# Autodesk Inventor assembly: fourbarintakebearing_MIR_MIR1_MIR1_MIR
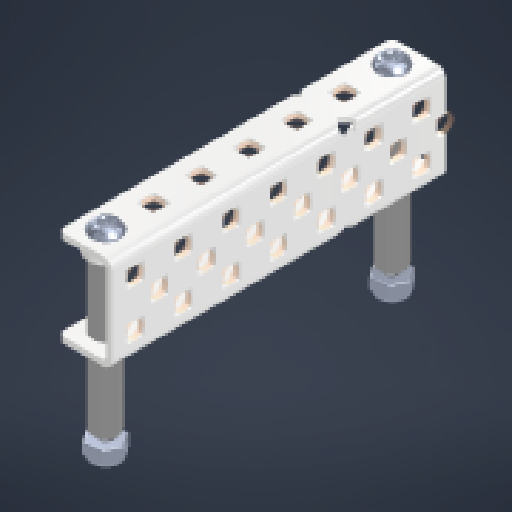
[picture p0: Inventor's stored thumbnail of the model, 512x512]
Saved by Autodesk Inventor 2023 (Build 270158000, 158)
## iProperties
Created: 2023-08-08
Part Number: fourbarintakebearing_MIR_MIR1_MIR1_MIR
Document SubType Name: Assembly
Designer: srbel
Author: srbel
## Documents named in this file (9)
- C:\CAD\OverUnderCAD\Drive\fourbarintakebearing_MIR_MIR1_MIR1_MIR.iam
- C:\CAD\OverUnderCAD\VEX-CAD-Inventor-1.4.0\Structure\C Channel\Aluminum 1x2x1\Alu C 1x2x1x7_MIR_MIR1_MIR1_MIR.ipt
- C:\CAD\OverUnderCAD\VEX-CAD-Inventor-1.4.0\Structure\Standoff.ipt
- C:\CAD\OverUnderCAD\VEX-CAD-Inventor-1.4.0\Motion\Spacers\Spacer Nylon .313 OD\NSpacer .313 OD x .125.ipt
- C:\CAD\OverUnderCAD\VEX-CAD-Inventor-1.4.0\Motion\Spacers\Spacer Nylon .313 OD.ipt
- C:\CAD\OverUnderCAD\VEX-CAD-Inventor-1.4.0\Structure\Standoff\Standoff .75.ipt
- C:\CAD\OverUnderCAD\VEX-CAD-Inventor-1.4.0\Structure\Hardware\Screw Steel - Star\SScrew Star Threaded 1.750.ipt
- C:\CAD\OverUnderCAD\VEX-CAD-Inventor-1.4.0\Structure\Hardware\Screw Steel - Star.ipt
- C:\CAD\OverUnderCAD\VEX-CAD-Inventor-1.4.0\Structure\Hardware\Nut Thin Nylock_MIR7_MIR1_MIR1_MIR.ipt
## Components (11 placed, 5 different names)
1. Alu C 1x2x1x7_MIR_MIR1_MIR1_MIR:1 — Insert:4, Insert:6, Insert:9, Insert:12, Insert:11, Insert:12
2. NSpacer .313 OD x .125:1 — Insert:4, Insert:3
3. Standoff .75:3 — Insert:3
4. NSpacer .313 OD x .125:2 — Insert:6, Insert:5
5. Standoff .75:4 — Insert:5
6. SScrew Star Threaded 1.750:1 — Insert:9
7. SScrew Star Threaded 1.750:2 — Insert:12
8. Standoff .75:5 — Insert:11, Insert:13
9. Standoff .75:6 — Insert:12, Insert:14
10. Nut Thin Nylock_MIR7_MIR1_MIR1_MIR:1 — Insert:13
11. Nut Thin Nylock_MIR7_MIR1_MIR1_MIR:2 — Insert:14
## Relationships (10: Insert 10)
- Insert:4: Alu C 1x2x1x7_MIR_MIR1_MIR1_MIR:1 ↔ NSpacer .313 OD x .125:1
- Insert:3: NSpacer .313 OD x .125:1 ↔ Standoff .75:3
- Insert:6: Alu C 1x2x1x7_MIR_MIR1_MIR1_MIR:1 ↔ NSpacer .313 OD x .125:2
- Insert:5: NSpacer .313 OD x .125:2 ↔ Standoff .75:4
- Insert:9: Alu C 1x2x1x7_MIR_MIR1_MIR1_MIR:1 ↔ SScrew Star Threaded 1.750:1
- Insert:12: Alu C 1x2x1x7_MIR_MIR1_MIR1_MIR:1 ↔ SScrew Star Threaded 1.750:2
- Insert:11: Alu C 1x2x1x7_MIR_MIR1_MIR1_MIR:1 ↔ Standoff .75:5
- Insert:12: Alu C 1x2x1x7_MIR_MIR1_MIR1_MIR:1 ↔ Standoff .75:6
- Insert:13 (1.5875 mm): Standoff .75:5 ↔ Nut Thin Nylock_MIR7_MIR1_MIR1_MIR:1
- Insert:14 (1.5875 mm): Standoff .75:6 ↔ Nut Thin Nylock_MIR7_MIR1_MIR1_MIR:2
